# Autodesk Inventor assembly: DCMotors_MockupAssm
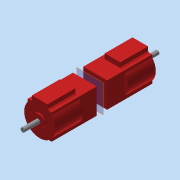
[picture p0: Inventor's stored thumbnail of the model, 180x180]
Saved by Autodesk Inventor 2016 (Build 200138000, 138)
## iProperties
Created: 2017-10-09
Part Number: DCMotors_MockupAssm
Document SubType Name: Assembly
Designer: rahul
Author: rahul
## Documents named in this file (3)
- C:\Users\rahul\Documents\Projects\BetaFish\Mechanical Design\DCMotors_MockupAssm.iam
- C:\Users\rahul\Documents\Projects\BetaFish\Mechanical Design\Jinlong_Z4TH5B1241992_VibrationMotor_NoWeight_Mockup.ipt
- C:\Users\rahul\Documents\Projects\BetaFish\Mechanical Design\Minebea_SMS6-20_StepperMotor_Mockup.ipt
## Components (4 placed, 2 different names)
1. Jinlong_Z4TH5B1241992_VibrationMotor_NoWeight_Mockup:1 — Flush:1, Flush:2, Flush:3, Mate:2, Mate:3, Mate:6, Flush:6
2. Jinlong_Z4TH5B1241992_VibrationMotor_NoWeight_Mockup:2 — Flush:1, Flush:2, Flush:4, Flush:5, Mate:5
3. Minebea_SMS6-20_StepperMotor_Mockup:1 — Flush:5, Mate:5, Flush:7
4. Minebea_SMS6-20_StepperMotor_Mockup:2 — Mate:6, Flush:6, Mate:7
## Relationships (13: Flush 7, Mate 6)
- Flush:1: Jinlong_Z4TH5B1241992_VibrationMotor_NoWeight_Mockup:1 ↔ Jinlong_Z4TH5B1241992_VibrationMotor_NoWeight_Mockup:2
- Flush:2: Jinlong_Z4TH5B1241992_VibrationMotor_NoWeight_Mockup:1 ↔ Jinlong_Z4TH5B1241992_VibrationMotor_NoWeight_Mockup:2
- Flush:3: Jinlong_Z4TH5B1241992_VibrationMotor_NoWeight_Mockup:1
- Mate:2: Jinlong_Z4TH5B1241992_VibrationMotor_NoWeight_Mockup:1
- Flush:4 (1 mm): Jinlong_Z4TH5B1241992_VibrationMotor_NoWeight_Mockup:2
- Mate:3 (1 mm): Jinlong_Z4TH5B1241992_VibrationMotor_NoWeight_Mockup:1
- Mate:4
- Flush:5: Jinlong_Z4TH5B1241992_VibrationMotor_NoWeight_Mockup:2 ↔ Minebea_SMS6-20_StepperMotor_Mockup:1
- Mate:5: Jinlong_Z4TH5B1241992_VibrationMotor_NoWeight_Mockup:2 ↔ Minebea_SMS6-20_StepperMotor_Mockup:1
- Mate:6: Jinlong_Z4TH5B1241992_VibrationMotor_NoWeight_Mockup:1 ↔ Minebea_SMS6-20_StepperMotor_Mockup:2
- Flush:6: Jinlong_Z4TH5B1241992_VibrationMotor_NoWeight_Mockup:1 ↔ Minebea_SMS6-20_StepperMotor_Mockup:2
- Flush:7: Minebea_SMS6-20_StepperMotor_Mockup:1
- Mate:7: Minebea_SMS6-20_StepperMotor_Mockup:2
